# Autodesk Inventor assembly: SampleClampingSystem
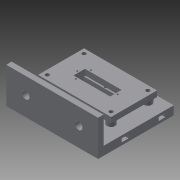
[picture p0: Inventor's stored thumbnail of the model, 180x180]
Saved by Autodesk Inventor 2015 (Build 190159000, 159)
## iProperties
Created: 2015-02-10
Part Number: SampleClampingSystem
Document SubType Name: Assembly
Designer: sgneitin
Author: sgneitin
## Documents named in this file (3)
- J:\ECEn 490\CAD\SampleClampingSystem\SampleClampingSystem.iam
- J:\ECEn 490\CAD\SampleClampingSystem\SampleBase.ipt
- J:\ECEn 490\CAD\SampleClampingSystem\490HV_MicrofluidicClamp.ipt
## Components (2 placed, 2 different names)
1. SampleBase:1 — Mate:1, Mate:2, Mate:3
2. 490HV_MicrofluidicClamp:1 — Mate:1, Mate:2, Mate:3
## Relationships (3: Mate 3)
- Mate:1: SampleBase:1 ↔ 490HV_MicrofluidicClamp:1
- Mate:2: SampleBase:1 ↔ 490HV_MicrofluidicClamp:1
- Mate:3 (1.27 mm): SampleBase:1 ↔ 490HV_MicrofluidicClamp:1
